# Autodesk Inventor assembly: wheel_molds_cut
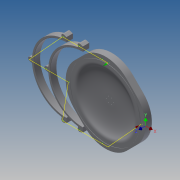
[picture p0: Inventor's stored thumbnail of the model, 180x180]
Saved by Autodesk Inventor 2015 (Build 190159000, 159)
## iProperties
Created: 2014-06-17
Part Number: wheel_molds_cut
Document SubType Name: Assembly
Designer: Yann
Author: Yann
## Documents named in this file (3)
- C:\Users\Yann\Documents\GitHub\Trike\Workspaces\Espace de travail\Source\Front_train\wheel_molds_cut.iam
- C:\Users\Yann\Documents\GitHub\Trike\Workspaces\Espace de travail\Source\Front_train\wheel_rim_mold_A.ipt
- C:\Users\Yann\Documents\GitHub\Trike\Workspaces\Espace de travail\Source\Front_train\wheel_rim_mold_B.ipt
## Components (3 placed, 2 different names)
1. wheel_rim_mold_A:1 — Mate:1, Mate:6, Mate:7, Mate:8
2. wheel_rim_mold_B:1 — Mate:3, Flush:8, Tangent:1
3. wheel_rim_mold_B:2 — Mate:2, Flush:7, Mate:8, Tangent:1
## Relationships (11: Mate 6, Flush 4, Tangent 1)
- Mate:1: wheel_rim_mold_A:1
- Mate:2: wheel_rim_mold_B:2
- Mate:3: wheel_rim_mold_B:1
- Flush:7: wheel_rim_mold_B:2
- Flush:8: wheel_rim_mold_B:1
- Mate:6: wheel_rim_mold_A:1
- Mate:7: wheel_rim_mold_A:1
- Mate:8 (14 mm): wheel_rim_mold_A:1 ↔ wheel_rim_mold_B:2
- Tangent:1 (12 mm): wheel_rim_mold_B:1 ↔ wheel_rim_mold_B:2
- Flush:9 (68.2625 mm)
- Flush:10 (-55.5625 mm)
